# Autodesk Inventor assembly: wing_MIR
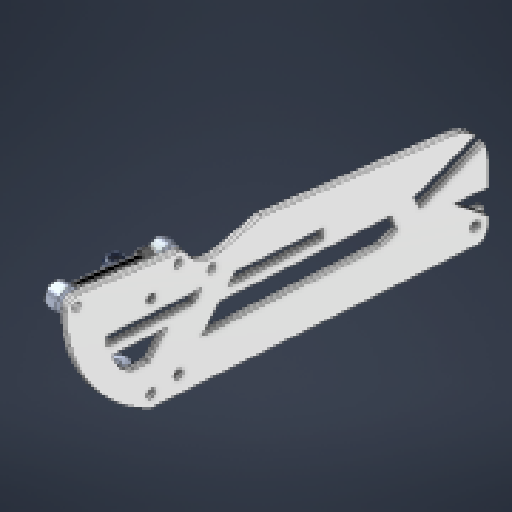
[picture p0: Inventor's stored thumbnail of the model, 512x512]
Saved by Autodesk Inventor 2024 (Build 280153000, 153)
## iProperties
Created: 2023-11-03
Part Number: wing_MIR
Document SubType Name: Assembly
Designer: avere
Author: avere
## Documents named in this file (12)
- C:\Users\avere\Documents\rbp_cad\zoomba_v0.1\chassis\wing\wing_MIR.iam
- C:\Users\avere\Documents\rbp_cad\zoomba_v0.1\chassis\wing\sled_MIR.ipt
- C:\Users\avere\Documents\rbp_cad\zoomba_v0.1\chassis\wing\Shaft Collar No Screw_MIR.ipt
- C:\Users\avere\Documents\rbp_cad\zoomba_v0.1\chassis\wing\Nut Thin Nylock_MIR.ipt
- C:\Users\avere\Documents\rbp_cad\zoomba_v0.1\chassis\wing\Alu Angle 1x1x12_MIR.ipt
- C:\Users\avere\Documents\rbp_cad\VEX-CAD-Inventor-1.41\Motion\Spacers\Spacer Nylon .375 OD\NSpacer .375 OD x .125.ipt
- C:\Users\avere\Documents\rbp_cad\VEX-CAD-Inventor-1.41\Motion\Spacers\Spacer Nylon .375 OD.ipt
- C:\Users\avere\Documents\rbp_cad\zoomba_v0.1\chassis\wing\Standoff 1.25_MIR.ipt
- C:\Users\avere\Documents\rbp_cad\VEX-CAD-Inventor-1.41\Motion\Spacers\Washer Teflon\TWasher .375 OD x .04000.ipt
- C:\Users\avere\Documents\rbp_cad\VEX-CAD-Inventor-1.41\Motion\Spacers\Washer Teflon.ipt
- C:\Users\avere\Documents\rbp_cad\VEX-CAD-Inventor-1.41\Motion\Spacers\Spacer Nylon .375 OD\NSpacer .375 OD x .375.ipt
- C:\Users\avere\Documents\rbp_cad\zoomba_v0.1\chassis\custom_parts\sled.ipt
## Components (13 placed, 9 different names)
1. sled_MIR:1 — Insert:11, Mate:5, Insert:15, Mate:4, Insert:10, Insert:16, Insert:17, Insert:11, Mate:5
2. Shaft Collar No Screw_MIR:1 — Insert:11, Insert:9
3. Shaft Collar No Screw_MIR:2 — Insert:9, Insert:8, Mate:6
4. Shaft Collar No Screw_MIR:3 — Mate:5, Mate:3
5. Shaft Collar No Screw_MIR:4 — Insert:15, Mate:3, Insert:14
6. Nut Thin Nylock_MIR:1 — Insert:8
7. Alu Angle 1x1x12_MIR:1 — Mate:4, Insert:10
8. NSpacer .375 OD x .125:1 — Insert:13, Insert:12
9. Standoff 1.25_MIR:1 — Insert:13
10. TWasher .375 OD x .04000:1 — Insert:14, Insert:12
11. NSpacer .375 OD x .375:2 — Mate:6, Insert:16
12. NSpacer .375 OD x .375:3 — Insert:17
13. sled:1 — Insert:11, Mate:5
## Relationships (16: Insert 11, Mate 5)
- Insert:11 (10.3188 mm): sled_MIR:1 ↔ Shaft Collar No Screw_MIR:1
- Insert:9 (34.925 mm): Shaft Collar No Screw_MIR:1 ↔ Shaft Collar No Screw_MIR:2
- Mate:5: sled_MIR:1 ↔ Shaft Collar No Screw_MIR:3
- Insert:15 (1.5875 mm): sled_MIR:1 ↔ Shaft Collar No Screw_MIR:4
- Mate:3: Shaft Collar No Screw_MIR:3 ↔ Shaft Collar No Screw_MIR:4
- Insert:8: Shaft Collar No Screw_MIR:2 ↔ Nut Thin Nylock_MIR:1
- Mate:4: sled_MIR:1 ↔ Alu Angle 1x1x12_MIR:1
- Insert:10: sled_MIR:1 ↔ Alu Angle 1x1x12_MIR:1
- Insert:13: NSpacer .375 OD x .125:1 ↔ Standoff 1.25_MIR:1
- Insert:14: Shaft Collar No Screw_MIR:4 ↔ TWasher .375 OD x .04000:1
- Insert:12: NSpacer .375 OD x .125:1 ↔ TWasher .375 OD x .04000:1
- Mate:6: Shaft Collar No Screw_MIR:2 ↔ NSpacer .375 OD x .375:2
- Insert:16: sled_MIR:1 ↔ NSpacer .375 OD x .375:2
- Insert:17: sled_MIR:1 ↔ NSpacer .375 OD x .375:3
- Insert:11: sled_MIR:1 ↔ sled:1
- Mate:5: sled_MIR:1 ↔ sled:1
